# Autodesk Inventor assembly: snowBlowerAndMount
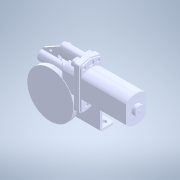
[picture p0: Inventor's stored thumbnail of the model, 180x180]
Saved by Autodesk Inventor 2022.1 (Build 261234020, 234B)
## iProperties
Created: 2021-11-10
Part Number: snowBlowerAndMount
Document SubType Name: Assembly
Designer: robst
Author: robst
## Documents named in this file (3)
- C:\git\CAD-Development\robSteele\snowBlowerAndMount.iam
- C:\git\CAD-MfgResources\Andy-Mark\MotorMounts\am-2373 Snow Blower Motor Mount.ipt
- C:\git\CAD-MfgResources\Andy-Mark\Motors\SnowBlowerMotor\AM-2235.iam
## Components (2 placed, 2 different names)
1. am-2373 Snow Blower Motor Mount:1 — Insert:2, Insert:3
2. AM-2235:1 [sub-assembly] — Insert:2, Insert:3
## Relationships (2: Insert 2)
- Insert:2: am-2373 Snow Blower Motor Mount:1 ↔ AM-2235:1
- Insert:3: am-2373 Snow Blower Motor Mount:1 ↔ AM-2235:1
